# Autodesk Inventor assembly: FreeBOT_mechanism
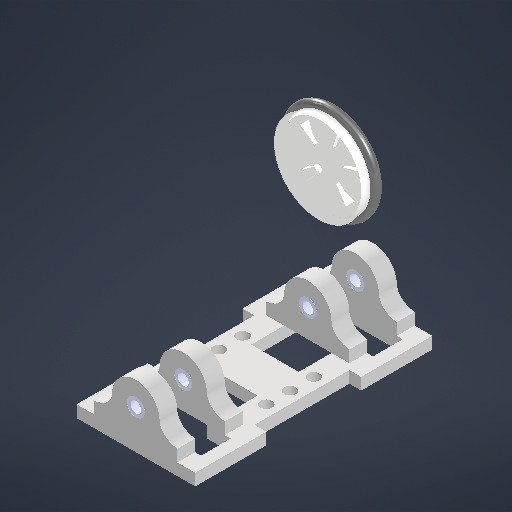
[picture p0: Inventor's stored thumbnail of the model, 512x512]
Saved by Autodesk Inventor 2027 (Build 310192060, 192F)
## iProperties
Created: 2026-07-01
Part Number: FreeBOT_mechanism
Document SubType Name: Assembly
Designer: loren
Author: loren
## Documents named in this file (6)
- C:\Users\loren\Desktop\Tesi Magistrale\CAD\FreeBOT\FreeBOT_mechanism.iam
- C:\Users\loren\Desktop\Tesi Magistrale\CAD\FreeBOT\chassis.ipt
- C:\Users\loren\Desktop\Tesi Magistrale\CAD\BB8\轮子1\轮子1.ipt
- C:\Users\loren\Desktop\Tesi Magistrale\CAD\BB8\初装\轮胎1.ipt
- C:\Users\loren\Desktop\Tesi Magistrale\CAD\BB8\初装\铜套.ipt
- C:\Users\loren\Desktop\Tesi Magistrale\CAD\FreeBOT\chassis 2.ipt
## Components (11 placed, 5 different names)
1. chassis:1 — Rigid:1, Mate:1, Mate:2, Mate:3, Rigid:5, Rigid:6, Rigid:7
2. chassis 2:1 — Rigid:1, Mate:1, Mate:2, Mate:3, Cylindrical:1
3. 轮子1:2 — Rigid:4
4. 轮胎1:3 — Rigid:4
5. chassis 2:2 — Rigid:7, Rigid:10
6. chassis 2:3 — Rigid:6, Rigid:9
7. chassis 2:4 — Rigid:5, Rigid:8
8. 铜套:1 — Cylindrical:1
9. 铜套:2 — Rigid:8
10. 铜套:3 — Rigid:9
11. 铜套:4 — Rigid:10
## Relationships (12: WeldJoint 8, Mate 3, CylindricalJoint 1)
- Rigid:1 [WeldJoint]: chassis:1 ↔ chassis 2:1
- Rigid:4 [WeldJoint] (1.5875 mm): 轮子1:2 ↔ 轮胎1:3
- Mate:1: chassis:1 ↔ chassis 2:1
- Mate:2: chassis:1 ↔ chassis 2:1
- Mate:3: chassis:1 ↔ chassis 2:1
- Rigid:5 [WeldJoint]: chassis:1 ↔ chassis 2:4
- Rigid:6 [WeldJoint]: chassis:1 ↔ chassis 2:3
- Rigid:7 [WeldJoint]: chassis:1 ↔ chassis 2:2
- Cylindrical:1: chassis 2:1 ↔ 铜套:1
- Rigid:8 [WeldJoint]: chassis 2:4 ↔ 铜套:2
- Rigid:9 [WeldJoint]: chassis 2:3 ↔ 铜套:3
- Rigid:10 [WeldJoint]: chassis 2:2 ↔ 铜套:4
